# Autodesk Inventor assembly: RobotConceptTesting2
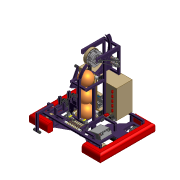
[picture p0: Inventor's stored thumbnail of the model, 180x180]
Saved by Autodesk Inventor 2012 (Build 160160000, 160)
## iProperties
Created: 2012-01-20
Part Number: RobotConceptTesting2
Document SubType Name: Assembly
Designer: JesseK
Mass: 36861.4 g
Surface Area: 274192 cm^2
Volume: 35910.7 cm^3
Density: 1.02648 g/cm^3
Author: JesseK
## Documents named in this file (12)
- Z:\UserData\Documents\Inventor\team1885frc\Robot2012\RobotConceptTesting2.iam
- Z:\UserData\Documents\Inventor\team1885frc\Robot2012\Concepts\Floor.ipt
- Z:\UserData\Documents\Inventor\team1885frc\Robot2012\DriveTrain\DiveTrain_FullAssembly.iam
- Z:\UserData\Documents\Inventor\team1885frc\Robot2012\ConveyorBaseAssembly.iam
- Z:\UserData\Documents\Inventor\team1885frc\Robot2012\Conveyor3\Conveyor3_FullAssembly.iam
- Z:\UserData\Documents\Inventor\team1885frc\Field\Compressed ball.ipt
- Z:\UserData\Documents\Inventor\team1885frc\Electronics\Battery.ipt
- Z:\UserData\Documents\Inventor\team1885frc\Robot2012\Electronics Board\Board_Final.iam
- Z:\UserData\Documents\Inventor\team1885frc\Banebots\RS-550_Assembly.iam
- Z:\UserData\Documents\Inventor\team1885frc\Robot2012\BridgeLoweringDevice\BridgeLoweringDeviceAssembly.iam
- Z:\UserData\Documents\Inventor\team1885frc\Robot2012\Bumpers_Red.ipt
- Z:\UserData\Documents\Inventor\team1885frc\Robot2012\Shroud.ipt
## Components (16 placed, 11 different names)
1. Floor:1 — Mate:1, Mate:35
2. DiveTrain_FullAssembly:1 [sub-assembly] — Mate:1, Mate:2, Flush:3, Mate:19, Mate:22, Mate:23, Mate:27, Mate:28, Mate:29, Mate:30, Mate:31, Mate:32, Mate:33
3. ConveyorBaseAssembly:1 [sub-assembly] — Mate:2, Flush:3, Flush:5, Mate:6, Mate:14, Mate:19, Flush:10, Mate:24, Mate:26, Flush:11, Flush:12, Tangent:1, Tangent:3, Tangent:5
4. Conveyor3_FullAssembly:1 [sub-assembly] — Flush:5, Mate:6, Mate:14, Mate:20, Mate:21, Mate:25, Mate:37, Tangent:2, Tangent:4, Tangent:6
5. Compressed ball:1 — Tangent:1, Tangent:2
6. Compressed ball:2 — Tangent:3, Tangent:4
7. Compressed ball:3 — Tangent:5, Tangent:6
8. Compressed ball:4
9. Battery:1 — Mate:22, Mate:23, Mate:24
10. Board_Final:1 [sub-assembly] — Flush:10, Mate:20, Mate:21, Mate:36, Flush:13
11. RS-550_Assembly:1 [sub-assembly] — Mate:26, Flush:11
12. RS-550_Assembly:2 [sub-assembly] — Mate:25, Flush:12
13. BridgeLoweringDeviceAssembly:1 [sub-assembly] — Mate:27, Mate:28, Mate:29
14. Bumpers_Red:1 — Mate:30, Mate:32, Mate:34
15. Bumpers_Red:2 — Mate:31, Mate:33, Mate:34, Mate:35
16. Shroud:1 — Mate:36, Flush:13, Mate:37
## Relationships (35: Mate 23, Flush 6, Tangent 6)
- Mate:1 (88.9 mm): Floor:1 ↔ DiveTrain_FullAssembly:1
- Mate:2: DiveTrain_FullAssembly:1 ↔ ConveyorBaseAssembly:1
- Flush:3: DiveTrain_FullAssembly:1 ↔ ConveyorBaseAssembly:1
- Flush:5: ConveyorBaseAssembly:1 ↔ Conveyor3_FullAssembly:1
- Mate:6: ConveyorBaseAssembly:1 ↔ Conveyor3_FullAssembly:1
- Mate:14: ConveyorBaseAssembly:1 ↔ Conveyor3_FullAssembly:1
- Mate:19: DiveTrain_FullAssembly:1 ↔ ConveyorBaseAssembly:1
- Flush:10: ConveyorBaseAssembly:1 ↔ Board_Final:1
- Mate:20: Conveyor3_FullAssembly:1 ↔ Board_Final:1
- Mate:21: Conveyor3_FullAssembly:1 ↔ Board_Final:1
- Mate:22: DiveTrain_FullAssembly:1 ↔ Battery:1
- Mate:23: DiveTrain_FullAssembly:1 ↔ Battery:1
- Mate:24: ConveyorBaseAssembly:1 ↔ Battery:1
- Mate:25: Conveyor3_FullAssembly:1 ↔ RS-550_Assembly:2
- Mate:26: ConveyorBaseAssembly:1 ↔ RS-550_Assembly:1
- Flush:11: ConveyorBaseAssembly:1 ↔ RS-550_Assembly:1
- Flush:12: ConveyorBaseAssembly:1 ↔ RS-550_Assembly:2
- Mate:27: DiveTrain_FullAssembly:1 ↔ BridgeLoweringDeviceAssembly:1
- Mate:28 (12.7 mm): DiveTrain_FullAssembly:1 ↔ BridgeLoweringDeviceAssembly:1
- Mate:29: DiveTrain_FullAssembly:1 ↔ BridgeLoweringDeviceAssembly:1
- Mate:30: DiveTrain_FullAssembly:1 ↔ Bumpers_Red:1
- Mate:31: DiveTrain_FullAssembly:1 ↔ Bumpers_Red:2
- Mate:32: DiveTrain_FullAssembly:1 ↔ Bumpers_Red:1
- Mate:33: DiveTrain_FullAssembly:1 ↔ Bumpers_Red:2
- Mate:34: Bumpers_Red:1 ↔ Bumpers_Red:2
- Mate:35 (50.8 mm): Floor:1 ↔ Bumpers_Red:2
- Mate:36: Board_Final:1 ↔ Shroud:1
- Flush:13: Board_Final:1 ↔ Shroud:1
- Mate:37: Conveyor3_FullAssembly:1 ↔ Shroud:1
- Tangent:1: ConveyorBaseAssembly:1 ↔ Compressed ball:1
- Tangent:2: Conveyor3_FullAssembly:1 ↔ Compressed ball:1
- Tangent:3: ConveyorBaseAssembly:1 ↔ Compressed ball:2
- Tangent:4: Conveyor3_FullAssembly:1 ↔ Compressed ball:2
- Tangent:5: ConveyorBaseAssembly:1 ↔ Compressed ball:3
- Tangent:6: Conveyor3_FullAssembly:1 ↔ Compressed ball:3
